# Autodesk Inventor assembly: finalthinksoomodule2
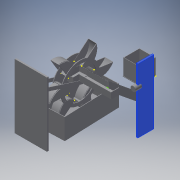
[picture p0: Inventor's stored thumbnail of the model, 180x180]
Saved by Autodesk Inventor 2019 (Build 230136000, 136)
## iProperties
Created: 2020-03-04
Part Number: finalthinksoomodule2
Document SubType Name: Assembly
Designer: Lenovo
Author: Lenovo
## Documents named in this file (10)
- C:\Users\Lenovo\Documents\finalthinksoomodule2.iam
- C:\Users\Lenovo\Documents\stand n wheel.iam
- C:\Users\Lenovo\Documents\holder2.ipt
- C:\Users\Lenovo\Documents\sidestandthroghdown.ipt
- C:\Users\Lenovo\Documents\elevation.ipt
- C:\Users\Lenovo\Documents\remainedpart.ipt
- C:\Users\Lenovo\Documents\wallforgarnishing.ipt
- C:\Users\Lenovo\Documents\garnishing.ipt
- C:\Users\Lenovo\Documents\garnishingslap.ipt
- E:\exploration\o2[930].ipt
## Components (9 placed, 9 different names)
1. stand n wheel:1 [sub-assembly]
2. holder2:1
3. sidestandthroghdown:1
4. elevation:1
5. remainedpart:1
6. wallforgarnishing:1 — Mate:1, Mate:2
7. garnishing:1 — Mate:2, Rigid:1, Rigid:2
8. garnishingslap:1 — Rigid:1
9. o2[930]:1 — Rigid:2
## Relationships (4: Mate 2, WeldJoint 2)
- Mate:1: wallforgarnishing:1
- Mate:2: wallforgarnishing:1 ↔ garnishing:1
- Rigid:1 [WeldJoint]: garnishing:1 ↔ garnishingslap:1
- Rigid:2 [WeldJoint]: garnishing:1 ↔ o2[930]:1
